# Autodesk Inventor assembly: wheelassembly
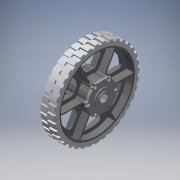
[picture p0: Inventor's stored thumbnail of the model, 180x180]
Saved by Autodesk Inventor 2019 (Build 230136000, 136)
## iProperties
Created: 2019-01-12
Part Number: wheelassembly
Document SubType Name: Assembly
Designer: lebraddock
Author: lebraddock
## Documents named in this file (3)
- C:\Users\lebraddock\Documents\CameronsRoboticsThings\2019 CAD\wheelassembly.iam
- C:\Users\lebraddock\Documents\CameronsRoboticsThings\2019 CAD\am-0940a 6 HiGrip wheel REV2.ipt
- C:\Users\lebraddock\Documents\CameronsRoboticsThings\2019 CAD\am-2568 500EX Hex Hub.ipt
## Components (3 placed, 2 different names)
1. am-0940a 6 HiGrip wheel REV2:1 — Mate:1, Mate:2, Mate:3, Mate:4
2. am-2568 500EX Hex Hub:1 — Mate:4, Flush:1, Flush:2
3. am-2568 500EX Hex Hub:2 — Mate:1, Mate:2, Mate:3, Flush:1, Flush:2
## Relationships (6: Mate 4, Flush 2)
- Mate:1: am-0940a 6 HiGrip wheel REV2:1 ↔ am-2568 500EX Hex Hub:2
- Mate:2: am-0940a 6 HiGrip wheel REV2:1 ↔ am-2568 500EX Hex Hub:2
- Mate:3: am-0940a 6 HiGrip wheel REV2:1 ↔ am-2568 500EX Hex Hub:2
- Mate:4: am-0940a 6 HiGrip wheel REV2:1 ↔ am-2568 500EX Hex Hub:1
- Flush:1: am-2568 500EX Hex Hub:1 ↔ am-2568 500EX Hex Hub:2
- Flush:2: am-2568 500EX Hex Hub:1 ↔ am-2568 500EX Hex Hub:2
